# Autodesk Inventor assembly: chain
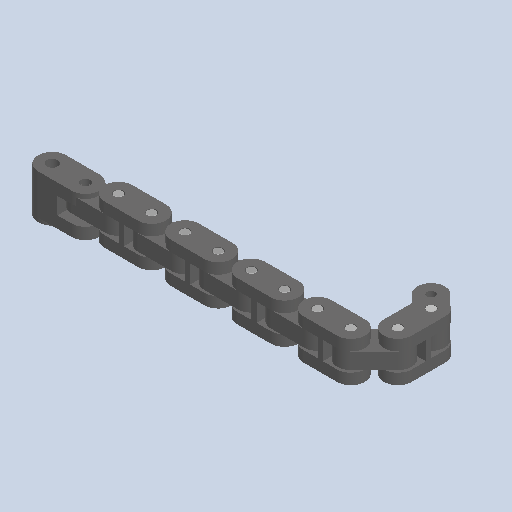
[picture p0: Inventor's stored thumbnail of the model, 512x512]
Saved by Autodesk Inventor 2024.1 (Build 281209000, 209)
## iProperties
Created: 2025-01-18
Part Number: chain
Document SubType Name: Assembly
Designer: hibik
Author: hibik
## Documents named in this file (5)
- C:\Users\hibik\Documents\Robomech\RESCUE\ORCA\hard\fork\right\chain.iam
- C:\Users\hibik\Documents\Robomech\RESCUE\ORCA\hard\fork\right\chain_1.ipt
- C:\Users\hibik\Documents\Robomech\RESCUE\ORCA\hard\fork\right\chain_2.ipt
- C:\Users\hibik\Documents\Robomech\RESCUE\ORCA\hard\std_parts\shaft_2_10.ipt
- C:\Users\hibik\Documents\Robomech\RESCUE\ORCA\hard\fork\right\chain_fork_connector.ipt
## Components (22 placed, 4 different names)
1. chain_2:4 — 角度:4, フラッシュ:12, 角度:8, メイト:1
2. chain_1:5 — 挿入:24, 挿入:32, 角度:4, 角度:5
3. shaft_2_10:5
4. chain_2:5 — 挿入:24, 角度:5, 角度:6
5. chain_1:6 — 挿入:25, 挿入:33, 角度:6, 角度:7, フラッシュ:5
6. shaft_2_10:6
7. chain_2:6 — 挿入:25, 角度:7, フラッシュ:6
8. chain_1:7 — 挿入:26, 挿入:34, フラッシュ:5, フラッシュ:7
9. shaft_2_10:7
10. chain_2:7 — 挿入:26, フラッシュ:6, フラッシュ:8
11. chain_1:8 — 挿入:27, 挿入:35, フラッシュ:7, フラッシュ:9
12. shaft_2_10:8
13. chain_2:8 — 挿入:27, フラッシュ:8, フラッシュ:10
14. chain_1:9 — 挿入:28, 挿入:36, フラッシュ:9, フラッシュ:13
15. shaft_2_10:9
16. chain_2:9 — 挿入:28, フラッシュ:10, 挿入:37
17. shaft_2_10:14 — 挿入:32
18. shaft_2_10:15 — 挿入:33
19. shaft_2_10:16 — 挿入:34
20. shaft_2_10:17 — 挿入:35
21. shaft_2_10:18 — 挿入:36
22. chain_fork_connector:1 — 挿入:37, フラッシュ:13
## Relationships (35: Insert 21, Flush 8, Angle 5, Mate 1)
- [Insert] (0.1 mm): chain_2:4 ↔ chain_1:5
- [Insert]: chain_1:5 ↔ shaft_2_10:5
- [Insert] (0.1 mm): chain_2:5 ↔ chain_1:6
- [Insert]: chain_1:6 ↔ shaft_2_10:6
- [Insert] (0.1 mm): chain_2:6 ↔ chain_1:7
- [Insert]: chain_1:7 ↔ shaft_2_10:7
- [Insert] (0.1 mm): chain_2:7 ↔ chain_1:8
- [Insert]: chain_1:8 ↔ shaft_2_10:8
- [Insert] (0.1 mm): chain_2:8 ↔ chain_1:9
- [Insert]: chain_1:9 ↔ shaft_2_10:9
- 挿入:24 [Insert] (0.1 mm): chain_1:5 ↔ chain_2:5
- 挿入:25 [Insert] (0.1 mm): chain_1:6 ↔ chain_2:6
- 挿入:26 [Insert] (0.1 mm): chain_1:7 ↔ chain_2:7
- 挿入:27 [Insert] (0.1 mm): chain_1:8 ↔ chain_2:8
- 挿入:28 [Insert] (0.1 mm): chain_1:9 ↔ chain_2:9
- 挿入:32 [Insert]: chain_1:5 ↔ shaft_2_10:14
- 挿入:33 [Insert]: chain_1:6 ↔ shaft_2_10:15
- 挿入:34 [Insert]: chain_1:7 ↔ shaft_2_10:16
- 挿入:35 [Insert]: chain_1:8 ↔ shaft_2_10:17
- 挿入:36 [Insert]: chain_1:9 ↔ shaft_2_10:18
- 角度:4 [Angle] (-45 deg): chain_2:4 ↔ chain_1:5
- 角度:5 [Angle] (-45 deg): chain_1:5 ↔ chain_2:5
- 角度:6 [Angle] (-45 deg): chain_2:5 ↔ chain_1:6
- 角度:7 [Angle] (0 deg): chain_1:6 ↔ chain_2:6
- フラッシュ:5 [Flush]: chain_1:6 ↔ chain_1:7
- フラッシュ:6 [Flush]: chain_2:6 ↔ chain_2:7
- フラッシュ:7 [Flush]: chain_1:7 ↔ chain_1:8
- フラッシュ:8 [Flush]: chain_2:7 ↔ chain_2:8
- フラッシュ:9 [Flush]: chain_1:8 ↔ chain_1:9
- フラッシュ:10 [Flush]: chain_2:8 ↔ chain_2:9
- フラッシュ:12 [Flush]: chain_2:4
- 角度:8 [Angle] (45 deg): chain_2:4
- 挿入:37 [Insert] (0.1 mm): chain_2:9 ↔ chain_fork_connector:1
- メイト:1 [Mate]: chain_2:4
- フラッシュ:13 [Flush]: chain_1:9 ↔ chain_fork_connector:1
## Named parameters: d13_d2 = 0.1 mm, d14_d10 = 0 mm, d15_d2 = 0.1 mm, d16_d10 = 0 mm, d17_d2 = 0.1 mm, d18_d10 = 0 mm, d19_d2 = 0.1 mm, d20_d10 = 0 mm, d21_d2 = 0.1 mm, d22_d10 = 0 mm
